# Autodesk Inventor assembly: MotorPulley_ASM
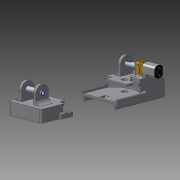
[picture p0: Inventor's stored thumbnail of the model, 180x180]
Saved by Autodesk Inventor 2014 SP1 (Build 180222100, 222)
## iProperties
Created: 2013-11-09
Part Number: MotorPulley_ASM
Document SubType Name: Assembly
Designer: JustinIndra
Author: JustinIndra
## Documents named in this file (7)
- C:\Users\JustinIndra\Dropbox\Projects\Mechatronics\Camera Slider\MotorizeKamerar\MECHANICAL\MotorPulley_ASM.iam
- C:\Users\JustinIndra\Dropbox\Projects\Mechatronics\Camera Slider\MotorizeKamerar\MECHANICAL\MotorHolder.ipt
- C:\Users\JustinIndra\Dropbox\Projects\Mechatronics\Camera Slider\MotorizeKamerar\MECHANICAL\PulleyHolder.ipt
- C:\Users\JustinIndra\Dropbox\Projects\Mechatronics\Camera Slider\MotorizeKamerar\MECHANICAL\PulleyShaft.ipt
- C:\Users\JustinIndra\Dropbox\Projects\Mechatronics\Camera Slider\MotorizeKamerar\MECHANICAL\MotorMount.ipt
- C:\Users\JustinIndra\Dropbox\Projects\Mechatronics\Camera Slider\MotorizeKamerar\MECHANICAL\ShaftConverter.ipt
- C:\Users\JustinIndra\Dropbox\Projects\Mechatronics\Camera Slider\MotorizeKamerar\MECHANICAL\OFF THE SHELF\Pololu #2218 Micro Metal Gearmotor HP.ipt
## Components (6 placed, 6 different names)
1. MotorHolder:1 — Flush:1, Flush:2, Mate:3, Mate:4, Mate:5, Mate:6, Mate:9
2. PulleyHolder:1 — Flush:1, Flush:2, Mate:2, Flush:3
3. PulleyShaft:1 — Mate:2, Flush:3
4. MotorMount:1 — Mate:3, Mate:4, Mate:5, Mate:7, Mate:8, Mate:10
5. ShaftConverter:1 — Mate:6, Mate:7
6. Pololu #2218 Micro Metal Gearmotor HP:1 — Mate:8, Mate:9, Mate:10
## Relationships (12: Mate 9, Flush 3)
- Flush:1: MotorHolder:1 ↔ PulleyHolder:1
- Flush:2: MotorHolder:1 ↔ PulleyHolder:1
- Mate:2: PulleyHolder:1 ↔ PulleyShaft:1
- Flush:3 (-1 mm): PulleyHolder:1 ↔ PulleyShaft:1
- Mate:3: MotorHolder:1 ↔ MotorMount:1
- Mate:4: MotorHolder:1 ↔ MotorMount:1
- Mate:5: MotorHolder:1 ↔ MotorMount:1
- Mate:6: MotorHolder:1 ↔ ShaftConverter:1
- Mate:7: MotorMount:1 ↔ ShaftConverter:1
- Mate:8: MotorMount:1 ↔ Pololu #2218 Micro Metal Gearmotor HP:1
- Mate:9: MotorHolder:1 ↔ Pololu #2218 Micro Metal Gearmotor HP:1
- Mate:10: MotorMount:1 ↔ Pololu #2218 Micro Metal Gearmotor HP:1
